# Autodesk Inventor assembly: BG201_trajan20_21
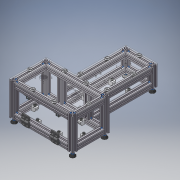
[picture p0: Inventor's stored thumbnail of the model, 180x180]
Saved by Autodesk Inventor 2022.2 (Build 262287000, 287)
## iProperties
Company: HTBLA Kaindorf
RuleStatus: InUse
Created: 2022-08-22
Part Number: BG201_trajan20_21
Project: Zeichenmaschine_v2
Material: Generisch
Description: gerüst_mit_platten
Document SubType Name: Assembly
Designer: trajan20
AfterDocNew0: iProperties-Editor_aufrufen
Author: jan
Keywords: 2021
## Documents named in this file (8)
- C:\Users\jan\Documents\DrawMachine\DrawMachineConstruction\Projekt\Zeichenmaschine_v2\BG201_trajan20_21_Zeichenmaschine_v2_gerüst_mit_platten.iam
- C:\Users\jan\Documents\DrawMachine\DrawMachineConstruction\Projekt\Zeichenmaschine_v2\BG103_trajan20_21_Zeichenmaschine_v2_Gerüst_Step_zu_Bauteil.iam
- C:\Users\jan\Documents\DrawMachine\DrawMachineConstruction\Projekt\Zeichenmaschine_v2\BT201_trajan20_21_Zeichenmaschine_v2_Hauptplatte unten.ipt
- C:\Users\jan\Documents\DrawMachine\DrawMachineConstruction\Projekt\Zeichenmaschine_v2\BT202_trajan20_21_Zeichenmaschine_v2_getriebemotor platte unten.ipt
- C:\Users\jan\Documents\DrawMachine\DrawMachineConstruction\Projekt\Zeichenmaschine_v2\BT101_trajan20_21_Zeichenmaschine_v2_Platte Stepper Motoren.ipt
- C:\Users\jan\Documents\DrawMachine\DrawMachineConstruction\Projekt\Zeichenmaschine_v2\BT102_trajan20_21_Zeichenmaschine_v2_Platte Getriebemotor.ipt
- C:\Users\jan\Documents\DrawMachine\DrawMachineConstruction\Projekt\Zeichenmaschine_v2\Normteile\de-DE\ISO 14583\ISO 14583 - M4x12-A3-70.ipt
- C:\Users\jan\Documents\DrawMachine\DrawMachineConstruction\Projekt\Zeichenmaschine_v2\step dateien\BN 603 1229915 finishing washer M5.ipt
## Components (27 placed, 7 different names)
1. BG103_trajan20_21_Zeichenmaschine_v2_Gerüst_Step_zu_Bauteil:1 [sub-assembly] — Passend:1, Passend:2, Passend:3, Passend:4, Passend:5, Passend:6, Passend:7, Fluchtend:1, Fluchtend:2, Fluchtend:3, Passend:8, Fluchtend:4
2. BT201_trajan20_21_Zeichenmaschine_v2_Hauptplatte unten:1 — Passend:1, Passend:2, Passend:3, Einfügen:1, Passend:9, Passend:10, Passend:11, Passend:12, Passend:13, Passend:14, Passend:15, Passend:16, Passend:17, Passend:18
3. BT202_trajan20_21_Zeichenmaschine_v2_getriebemotor platte unten:1 — Passend:4, Passend:5, Passend:6, Passend:19, Passend:20, Passend:21, Passend:22, Passend:23, Passend:24, Passend:25, Passend:26, Passend:27, Passend:28
4. BT101_trajan20_21_Zeichenmaschine_v2_Platte Stepper Motoren:1 — Passend:7, Fluchtend:1, Fluchtend:2, Passend:29, Passend:30, Passend:31, Passend:32, Passend:33, Passend:34, Passend:35, Passend:36, Passend:37, Passend:38, Passend:39, Passend:40
5. BT102_trajan20_21_Zeichenmaschine_v2_Platte Getriebemotor:1 — Fluchtend:3, Passend:8, Fluchtend:4, Passend:41, Passend:42, Passend:43, Passend:44, Passend:45, Passend:46, Passend:47, Passend:48, Passend:49, Passend:50
6. BN 603 1229915 finishing washer M5:1 — Passend:29, Passend:30
7. BN 603 1229915 finishing washer M5:2 — Passend:31, Passend:32
8. BN 603 1229915 finishing washer M5:3 — Passend:33, Passend:34
9. BN 603 1229915 finishing washer M5:4 — Passend:35, Passend:36
10. BN 603 1229915 finishing washer M5:5 — Passend:37, Passend:38
11. BN 603 1229915 finishing washer M5:6 — Passend:39, Passend:40
12. BN 603 1229915 finishing washer M5:7 — Passend:41, Passend:42
13. BN 603 1229915 finishing washer M5:8 — Passend:43, Passend:44
14. BN 603 1229915 finishing washer M5:9 — Passend:45, Passend:46
15. BN 603 1229915 finishing washer M5:10 — Passend:47, Passend:48
16. BN 603 1229915 finishing washer M5:11 — Passend:49, Passend:50
17. Schraube ISO 14583:2011(E) M4x12-A3-70:1 — Einfügen:1
18. Schraube ISO 14583:2011(E) M4x12-A3-70:2 — Passend:9, Passend:10
19. Schraube ISO 14583:2011(E) M4x12-A3-70:3 — Passend:11, Passend:12
20. Schraube ISO 14583:2011(E) M4x12-A3-70:4 — Passend:13, Passend:14
21. Schraube ISO 14583:2011(E) M4x12-A3-70:5 — Passend:15, Passend:16
22. Schraube ISO 14583:2011(E) M4x12-A3-70:6 — Passend:17, Passend:18
23. Schraube ISO 14583:2011(E) M4x12-A3-70:7 — Passend:19, Passend:20
24. Schraube ISO 14583:2011(E) M4x12-A3-70:8 — Passend:21, Passend:22
25. Schraube ISO 14583:2011(E) M4x12-A3-70:9 — Passend:23, Passend:24
26. Schraube ISO 14583:2011(E) M4x12-A3-70:10 — Passend:25, Passend:26
27. Schraube ISO 14583:2011(E) M4x12-A3-70:11 — Passend:27, Passend:28
## Relationships (55: Mate 50, Flush 4, Insert 1)
- Passend:1 [Mate]: BG103_trajan20_21_Zeichenmaschine_v2_Gerüst_Step_zu_Bauteil:1 ↔ BT201_trajan20_21_Zeichenmaschine_v2_Hauptplatte unten:1
- Passend:2 [Mate]: BG103_trajan20_21_Zeichenmaschine_v2_Gerüst_Step_zu_Bauteil:1 ↔ BT201_trajan20_21_Zeichenmaschine_v2_Hauptplatte unten:1
- Passend:3 [Mate]: BG103_trajan20_21_Zeichenmaschine_v2_Gerüst_Step_zu_Bauteil:1 ↔ BT201_trajan20_21_Zeichenmaschine_v2_Hauptplatte unten:1
- Passend:4 [Mate]: BG103_trajan20_21_Zeichenmaschine_v2_Gerüst_Step_zu_Bauteil:1 ↔ BT202_trajan20_21_Zeichenmaschine_v2_getriebemotor platte unten:1
- Passend:5 [Mate]: BG103_trajan20_21_Zeichenmaschine_v2_Gerüst_Step_zu_Bauteil:1 ↔ BT202_trajan20_21_Zeichenmaschine_v2_getriebemotor platte unten:1
- Passend:6 [Mate]: BG103_trajan20_21_Zeichenmaschine_v2_Gerüst_Step_zu_Bauteil:1 ↔ BT202_trajan20_21_Zeichenmaschine_v2_getriebemotor platte unten:1
- Passend:7 [Mate]: BG103_trajan20_21_Zeichenmaschine_v2_Gerüst_Step_zu_Bauteil:1 ↔ BT101_trajan20_21_Zeichenmaschine_v2_Platte Stepper Motoren:1
- Fluchtend:1 [Flush]: BG103_trajan20_21_Zeichenmaschine_v2_Gerüst_Step_zu_Bauteil:1 ↔ BT101_trajan20_21_Zeichenmaschine_v2_Platte Stepper Motoren:1
- Fluchtend:2 [Flush]: BG103_trajan20_21_Zeichenmaschine_v2_Gerüst_Step_zu_Bauteil:1 ↔ BT101_trajan20_21_Zeichenmaschine_v2_Platte Stepper Motoren:1
- Fluchtend:3 [Flush]: BG103_trajan20_21_Zeichenmaschine_v2_Gerüst_Step_zu_Bauteil:1 ↔ BT102_trajan20_21_Zeichenmaschine_v2_Platte Getriebemotor:1
- Passend:8 [Mate]: BG103_trajan20_21_Zeichenmaschine_v2_Gerüst_Step_zu_Bauteil:1 ↔ BT102_trajan20_21_Zeichenmaschine_v2_Platte Getriebemotor:1
- Fluchtend:4 [Flush]: BG103_trajan20_21_Zeichenmaschine_v2_Gerüst_Step_zu_Bauteil:1 ↔ BT102_trajan20_21_Zeichenmaschine_v2_Platte Getriebemotor:1
- Einfügen:1 [Insert]: BT201_trajan20_21_Zeichenmaschine_v2_Hauptplatte unten:1 ↔ Schraube ISO 14583:2011(E) M4x12-A3-70:1
- Passend:9 [Mate]: BT201_trajan20_21_Zeichenmaschine_v2_Hauptplatte unten:1 ↔ Schraube ISO 14583:2011(E) M4x12-A3-70:2
- Passend:10 [Mate]: BT201_trajan20_21_Zeichenmaschine_v2_Hauptplatte unten:1 ↔ Schraube ISO 14583:2011(E) M4x12-A3-70:2
- Passend:11 [Mate]: BT201_trajan20_21_Zeichenmaschine_v2_Hauptplatte unten:1 ↔ Schraube ISO 14583:2011(E) M4x12-A3-70:3
- Passend:12 [Mate]: BT201_trajan20_21_Zeichenmaschine_v2_Hauptplatte unten:1 ↔ Schraube ISO 14583:2011(E) M4x12-A3-70:3
- Passend:13 [Mate]: BT201_trajan20_21_Zeichenmaschine_v2_Hauptplatte unten:1 ↔ Schraube ISO 14583:2011(E) M4x12-A3-70:4
- Passend:14 [Mate]: BT201_trajan20_21_Zeichenmaschine_v2_Hauptplatte unten:1 ↔ Schraube ISO 14583:2011(E) M4x12-A3-70:4
- Passend:15 [Mate]: BT201_trajan20_21_Zeichenmaschine_v2_Hauptplatte unten:1 ↔ Schraube ISO 14583:2011(E) M4x12-A3-70:5
- Passend:16 [Mate]: BT201_trajan20_21_Zeichenmaschine_v2_Hauptplatte unten:1 ↔ Schraube ISO 14583:2011(E) M4x12-A3-70:5
- Passend:17 [Mate]: BT201_trajan20_21_Zeichenmaschine_v2_Hauptplatte unten:1 ↔ Schraube ISO 14583:2011(E) M4x12-A3-70:6
- Passend:18 [Mate]: BT201_trajan20_21_Zeichenmaschine_v2_Hauptplatte unten:1 ↔ Schraube ISO 14583:2011(E) M4x12-A3-70:6
- Passend:19 [Mate]: BT202_trajan20_21_Zeichenmaschine_v2_getriebemotor platte unten:1 ↔ Schraube ISO 14583:2011(E) M4x12-A3-70:7
- Passend:20 [Mate]: BT202_trajan20_21_Zeichenmaschine_v2_getriebemotor platte unten:1 ↔ Schraube ISO 14583:2011(E) M4x12-A3-70:7
- Passend:21 [Mate]: BT202_trajan20_21_Zeichenmaschine_v2_getriebemotor platte unten:1 ↔ Schraube ISO 14583:2011(E) M4x12-A3-70:8
- Passend:22 [Mate]: BT202_trajan20_21_Zeichenmaschine_v2_getriebemotor platte unten:1 ↔ Schraube ISO 14583:2011(E) M4x12-A3-70:8
- Passend:23 [Mate]: BT202_trajan20_21_Zeichenmaschine_v2_getriebemotor platte unten:1 ↔ Schraube ISO 14583:2011(E) M4x12-A3-70:9
- Passend:24 [Mate]: BT202_trajan20_21_Zeichenmaschine_v2_getriebemotor platte unten:1 ↔ Schraube ISO 14583:2011(E) M4x12-A3-70:9
- Passend:25 [Mate]: BT202_trajan20_21_Zeichenmaschine_v2_getriebemotor platte unten:1 ↔ Schraube ISO 14583:2011(E) M4x12-A3-70:10
- Passend:26 [Mate]: BT202_trajan20_21_Zeichenmaschine_v2_getriebemotor platte unten:1 ↔ Schraube ISO 14583:2011(E) M4x12-A3-70:10
- Passend:27 [Mate]: BT202_trajan20_21_Zeichenmaschine_v2_getriebemotor platte unten:1 ↔ Schraube ISO 14583:2011(E) M4x12-A3-70:11
- Passend:28 [Mate]: BT202_trajan20_21_Zeichenmaschine_v2_getriebemotor platte unten:1 ↔ Schraube ISO 14583:2011(E) M4x12-A3-70:11
- Passend:29 [Mate]: BT101_trajan20_21_Zeichenmaschine_v2_Platte Stepper Motoren:1 ↔ BN 603 1229915 finishing washer M5:1
- Passend:30 [Mate]: BT101_trajan20_21_Zeichenmaschine_v2_Platte Stepper Motoren:1 ↔ BN 603 1229915 finishing washer M5:1
- Passend:31 [Mate]: BT101_trajan20_21_Zeichenmaschine_v2_Platte Stepper Motoren:1 ↔ BN 603 1229915 finishing washer M5:2
- Passend:32 [Mate]: BT101_trajan20_21_Zeichenmaschine_v2_Platte Stepper Motoren:1 ↔ BN 603 1229915 finishing washer M5:2
- Passend:33 [Mate]: BT101_trajan20_21_Zeichenmaschine_v2_Platte Stepper Motoren:1 ↔ BN 603 1229915 finishing washer M5:3
- Passend:34 [Mate]: BT101_trajan20_21_Zeichenmaschine_v2_Platte Stepper Motoren:1 ↔ BN 603 1229915 finishing washer M5:3
- Passend:35 [Mate]: BT101_trajan20_21_Zeichenmaschine_v2_Platte Stepper Motoren:1 ↔ BN 603 1229915 finishing washer M5:4
- Passend:36 [Mate]: BT101_trajan20_21_Zeichenmaschine_v2_Platte Stepper Motoren:1 ↔ BN 603 1229915 finishing washer M5:4
- Passend:37 [Mate]: BT101_trajan20_21_Zeichenmaschine_v2_Platte Stepper Motoren:1 ↔ BN 603 1229915 finishing washer M5:5
- Passend:38 [Mate]: BT101_trajan20_21_Zeichenmaschine_v2_Platte Stepper Motoren:1 ↔ BN 603 1229915 finishing washer M5:5
- Passend:39 [Mate]: BT101_trajan20_21_Zeichenmaschine_v2_Platte Stepper Motoren:1 ↔ BN 603 1229915 finishing washer M5:6
- Passend:40 [Mate]: BT101_trajan20_21_Zeichenmaschine_v2_Platte Stepper Motoren:1 ↔ BN 603 1229915 finishing washer M5:6
- Passend:41 [Mate]: BT102_trajan20_21_Zeichenmaschine_v2_Platte Getriebemotor:1 ↔ BN 603 1229915 finishing washer M5:7
- Passend:42 [Mate]: BT102_trajan20_21_Zeichenmaschine_v2_Platte Getriebemotor:1 ↔ BN 603 1229915 finishing washer M5:7
- Passend:43 [Mate]: BT102_trajan20_21_Zeichenmaschine_v2_Platte Getriebemotor:1 ↔ BN 603 1229915 finishing washer M5:8
- Passend:44 [Mate]: BT102_trajan20_21_Zeichenmaschine_v2_Platte Getriebemotor:1 ↔ BN 603 1229915 finishing washer M5:8
- Passend:45 [Mate]: BT102_trajan20_21_Zeichenmaschine_v2_Platte Getriebemotor:1 ↔ BN 603 1229915 finishing washer M5:9
- Passend:46 [Mate]: BT102_trajan20_21_Zeichenmaschine_v2_Platte Getriebemotor:1 ↔ BN 603 1229915 finishing washer M5:9
- Passend:47 [Mate]: BT102_trajan20_21_Zeichenmaschine_v2_Platte Getriebemotor:1 ↔ BN 603 1229915 finishing washer M5:10
- Passend:48 [Mate]: BT102_trajan20_21_Zeichenmaschine_v2_Platte Getriebemotor:1 ↔ BN 603 1229915 finishing washer M5:10
- Passend:49 [Mate]: BT102_trajan20_21_Zeichenmaschine_v2_Platte Getriebemotor:1 ↔ BN 603 1229915 finishing washer M5:11
- Passend:50 [Mate]: BT102_trajan20_21_Zeichenmaschine_v2_Platte Getriebemotor:1 ↔ BN 603 1229915 finishing washer M5:11
